# Autodesk Inventor assembly: A2017_T3_02
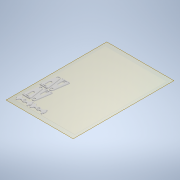
[picture p0: Inventor's stored thumbnail of the model, 180x180]
Saved by Autodesk Inventor 2020 (Build 240168000, 168)
## iProperties
Created: 2021-08-27
Part Number: A2017_T3_02
Document SubType Name: Assembly
Designer: Masato
Author: Masato
## Documents named in this file (4)
- C:\Users\naoki\Documents\Inventor\CitBrains\git_clone\OpenPlatform4_1\jig検証\OpenPlatform_ver3_0\cam\A2017_T3_02.iam
- C:\Users\naoki\Documents\Inventor\CitBrains\git_clone\OpenPlatform4_1\コックピット\OpenPlatform_ver3_0\cam\Disposable_Board.ipt
- C:\Users\naoki\Documents\Inventor\CitBrains\git_clone\OpenPlatform4_1\コックピット\OpenPlatform_ver3_0\LowerBody\Ankle\Ankle_front_frame.ipt
- C:\Users\naoki\Documents\Inventor\CitBrains\git_clone\OpenPlatform4_1\jig検証\OpenPlatform_ver3_0\LowerBody\Leg_joit\Leg_joint_slider_frame.ipt
## Components (7 placed, 3 different names)
1. Disposable_Board:1 — メイト:2, メイト:1, フラッシュ:1, フラッシュ:2, メイト:4, フラッシュ:3, フラッシュ:4, メイト:5, メイト:6, フラッシュ:5
2. Ankle_front_frame:1 — メイト:4, フラッシュ:3, フラッシュ:4, メイト:8
3. Ankle_front_frame:2
4. Leg_joint_slider_frame:1 — メイト:5, メイト:7, 正接:1, フラッシュ:5, メイト:8
5. Leg_joint_slider_frame:2 — メイト:6, メイト:7, 正接:1
6. Leg_joint_slider_frame:3
7. Leg_joint_slider_frame:4
## Component patterns: (2 elements, first: Ankle_front_frame:1), (2 elements, first: Leg_joint_slider_frame:1 + Leg_joint_slider_frame:2)
## Relationships (13: Mate 7, Flush 5, Tangent 1)
- メイト:2 [Mate]: Disposable_Board:1
- メイト:1 [Mate]: Disposable_Board:1
- フラッシュ:1 [Flush]: Disposable_Board:1
- フラッシュ:2 [Flush]: Disposable_Board:1
- メイト:4 [Mate]: Disposable_Board:1 ↔ Ankle_front_frame:1
- フラッシュ:3 [Flush] (2 mm): Disposable_Board:1 ↔ Ankle_front_frame:1
- フラッシュ:4 [Flush] (2 mm): Disposable_Board:1 ↔ Ankle_front_frame:1
- メイト:5 [Mate]: Disposable_Board:1 ↔ Leg_joint_slider_frame:1
- メイト:6 [Mate]: Disposable_Board:1 ↔ Leg_joint_slider_frame:2
- メイト:7 [Mate] (2.5 mm): Leg_joint_slider_frame:1 ↔ Leg_joint_slider_frame:2
- 正接:1 [Tangent]: Leg_joint_slider_frame:1 ↔ Leg_joint_slider_frame:2
- フラッシュ:5 [Flush] (2 mm): Disposable_Board:1 ↔ Leg_joint_slider_frame:1
- メイト:8 [Mate] (4 mm): Ankle_front_frame:1 ↔ Leg_joint_slider_frame:1
